# Autodesk Inventor assembly: EnCase
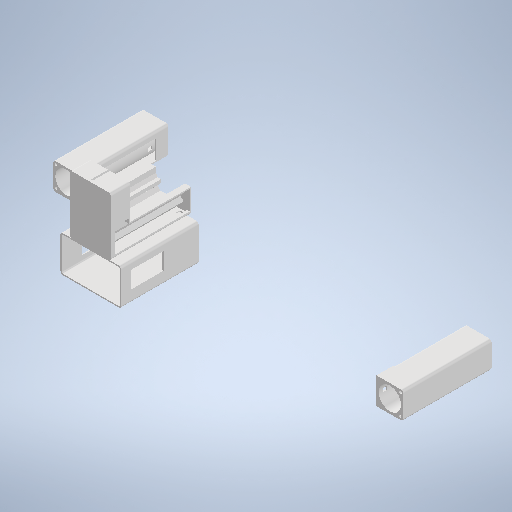
[picture p0: Inventor's stored thumbnail of the model, 512x512]
Saved by Autodesk Inventor 2025.2 (Build 292293000, 293)
## iProperties
Created: 2026-03-11
Part Number: EnCase
Document SubType Name: Assembly
Designer: Periscopio
Author: Periscopio
## Documents named in this file (5)
- C:\Users\Periscopio\Documents\SDV\Polígono\Diseño CAD\EnCase.iam
- C:\Users\Periscopio\Documents\SDV\Polígono\Diseño CAD\Box.ipt
- C:\Users\Periscopio\Documents\SDV\Polígono\Diseño CAD\Case.ipt
- C:\Users\Periscopio\Documents\SDV\Polígono\Diseño CAD\PortaPilasL.ipt
- C:\Users\Periscopio\Documents\SDV\Polígono\Diseño CAD\PortaPilasR.ipt
## Components (4 placed, 4 different names)
1. Box:1 — Coincidencia:1, Coincidencia:2, Coincidencia:3, Rígido:1
2. Case:1 — Coincidencia:1, Coincidencia:2, Coincidencia:3, Rígido:1
3. PortaPilasL:1
4. PortaPilasR:1
## Relationships (4: Mate 3, WeldJoint 1)
- Coincidencia:1 [Mate]: Box:1 ↔ Case:1
- Coincidencia:2 [Mate]: Box:1 ↔ Case:1
- Coincidencia:3 [Mate]: Box:1 ↔ Case:1
- Rígido:1 [WeldJoint]: Box:1 ↔ Case:1
